# Autodesk Inventor assembly: Working Encoder
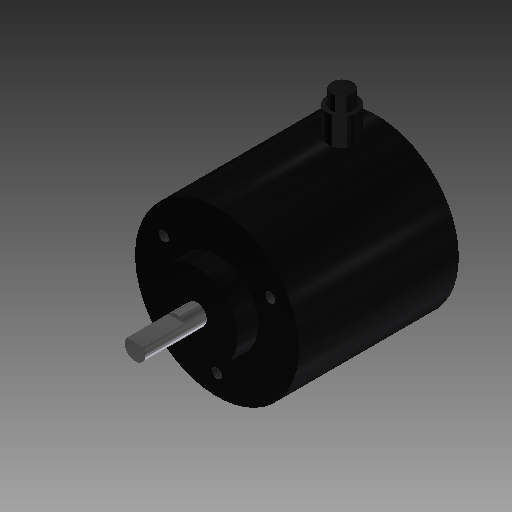
[picture p0: Inventor's stored thumbnail of the model, 512x512]
Saved by Autodesk Inventor 2018 (Build 220112000, 112)
## iProperties
Created: 2017-05-30
Part Number: Working Encoder
Document SubType Name: Assembly
Designer: M220404
Author: M220404
## Documents named in this file (3)
- C:\Users\P301319\Documents\GitHub\CNC-Lathe-CAD\CNC Lathe Project\Project Files\Encoder Subassembly\Working Encoder.iam
- C:\Users\P301319\Documents\GitHub\CNC-Lathe-CAD\CNC Lathe Project\Project Files\Encoder Subassembly\Belt Encoder Body.ipt
- C:\Users\P301319\Documents\GitHub\CNC-Lathe-CAD\CNC Lathe Project\Project Files\Encoder Subassembly\Belt encoder shaft.ipt
## Components (2 placed, 2 different names)
1. Belt Encoder Body:1 — Mate:1, Mate:2
2. Belt encoder shaft:1 — Mate:1, Mate:2
## Relationships (2: Mate 2)
- Mate:1: Belt Encoder Body:1 ↔ Belt encoder shaft:1
- Mate:2: Belt Encoder Body:1 ↔ Belt encoder shaft:1
